# Autodesk Inventor assembly: untitled.brd
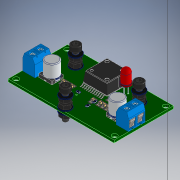
[picture p0: Inventor's stored thumbnail of the model, 180x180]
Saved by Autodesk Inventor 2022 (Build 260153000, 153)
## iProperties
Created: 2022-12-24
Part Number: untitled.brd
Document SubType Name: Assembly
Designer: Ivan Petrov
Author: Ivan Petrov
## Documents named in this file (12)
- C:\Users\Ivan Petrov\Documents\GitHub\OmniBot\design\000.007 - Бортовой источник питания СБ.iam
- C:\Users\Ivan Petrov\Documents\GitHub\OmniBot\design\000.007.001 - Плата печатная.ipt
- C:\Users\Ivan Petrov\Documents\GitHub\OmniBot\design\standart_components\TO-PMOD NDY-11.ipt
- C:\Users\Ivan Petrov\Documents\GitHub\OmniBot\design\standart_components\smd resistors\0R.iam
- C:\Users\Ivan Petrov\Documents\GitHub\OmniBot\design\standart_components\Capacitors smd\Сборка1.iam
- C:\Users\Ivan Petrov\Documents\GitHub\OmniBot\design\standart_components\Capacitors smd\05_NICHICON_8X10_NEWARK_58R3566_ENSAMBLE.ipt
- C:\Users\Ivan Petrov\Documents\GitHub\OmniBot\design\standart_components\LED-Red.ipt
- C:\Users\Ivan Petrov\Documents\GitHub\OmniBot\design\standart_components\Capacitors smd\000.007.002 - Радиатор.ipt
- C:\Users\Ivan Petrov\Documents\GitHub\OmniBot\design\standart_components\Terminal Block 2P.ipt
- C:\Users\Ivan Petrov\Documents\GitHub\OmniBot\design\Content Center Files\ru-RU\DIN 912\DIN 912 - M3 x 0,5 x 16 x 14,75.ipt
- C:\Users\Ivan Petrov\Documents\GitHub\OmniBot\design\Content Center Files\ru-RU\AS 1237 (3.1)\AS 1237 - 3 mm(1)Aluminium-6061.ipt
- C:\Users\Ivan Petrov\Documents\GitHub\OmniBot\design\Content Center Files\ru-RU\AS 1112 (2)\AS 1112 - M3  Тип 5.ipt
## Components (43 placed, 23 different names)
1. untitled.brdКонтур:1 — Совмещение:2, Совмещение:11, Совмещение:20, Совмещение:21, Совмещение:22, Совмещение:23, Совмещение:24, Совмещение:25, Угол:1, Совмещение:26, Угол:2, Вставка:4, Вставка:5, Вставка:6, Вставка:14, Вставка:15, Вставка:16
2. C1_2 [sub-assembly]
3. C2_3 [sub-assembly]
4. C3_4 [sub-assembly]
5. C4_5 [sub-assembly]
6. C5_6 [sub-assembly]
7. C6_7 [sub-assembly]
8. C7_8 [sub-assembly]
9. C8_9 [sub-assembly]
10. R1_24 [sub-assembly]
11. R2_25 [sub-assembly]
12. R3_26 [sub-assembly]
13. R4_27 [sub-assembly]
14. R5_28 [sub-assembly]
15. R6_29 [sub-assembly]
16. TO-PMOD NDY-11:1 — Совмещение:2, Заподлицо:1, Совмещение:27
17. 05_NICHICON_8X10_NEWARK_58R3566_ENSAMBLE:1 — Совмещение:10, Совмещение:11
18. 05_NICHICON_8X10_NEWARK_58R3566_ENSAMBLE:2 — Совмещение:19, Совмещение:20
19. LED-Red:1 — Совмещение:21, Совмещение:22, Заподлицо:1
20. 000.007.002 - Радиатор:1 — Совмещение:27, Вставка:1, Вставка:2, Вставка:3, Вставка:11, Вставка:12, Вставка:13
21. Terminal Block 2P:1 — Совмещение:23, Совмещение:25, Угол:1
22. Terminal Block 2P:2 — Совмещение:24, Совмещение:26, Угол:2
23. DIN 912 - заменено на DIN EN ISO 4762 M3 x 16:1 — Вставка:1
24. DIN 912 - заменено на DIN EN ISO 4762 M3 x 16:2 — Вставка:2
25. DIN 912 - заменено на DIN EN ISO 4762 M3 x 16:3 — Вставка:3
26. AS 1237 (3.1) 3 mm - Алюминий 6061:1 — Вставка:4, Вставка:19
27. AS 1237 (3.1) 3 mm - Алюминий 6061:2 — Вставка:5, Вставка:17
28. AS 1237 (3.1) 3 mm - Алюминий 6061:3 — Вставка:6, Вставка:18
29. AS 1237 (3.1) 3 mm - Алюминий 6061:8 — Вставка:11, Вставка:20
30. AS 1237 (3.1) 3 mm - Алюминий 6061:9 — Вставка:12, Вставка:21
31. AS 1237 (3.1) 3 mm - Алюминий 6061:10 — Вставка:13, Вставка:25
32. AS 1237 (3.1) 3 mm - Алюминий 6061:11 — Вставка:14, Вставка:23
33. AS 1237 (3.1) 3 mm - Алюминий 6061:12 — Вставка:15, Вставка:24
34. AS 1237 (3.1) 3 mm - Алюминий 6061:13 — Вставка:16, Вставка:22
35. AS 1112 (2) - метрическая M3  Тип 5:1 — Вставка:17
36. AS 1112 (2) - метрическая M3  Тип 5:2 — Вставка:18
37. AS 1112 (2) - метрическая M3  Тип 5:3 — Вставка:19
38. AS 1112 (2) - метрическая M3  Тип 5:4 — Вставка:20
39. AS 1112 (2) - метрическая M3  Тип 5:5 — Вставка:21
40. AS 1112 (2) - метрическая M3  Тип 5:6 — Вставка:22
41. AS 1112 (2) - метрическая M3  Тип 5:7 — Вставка:23
42. AS 1112 (2) - метрическая M3  Тип 5:8 — Вставка:24
43. AS 1112 (2) - метрическая M3  Тип 5:9 — Вставка:25
## Relationships (42: Insert 21, Mate 18, Angle 2, Flush 1)
- Совмещение:2 [Mate]: untitled.brdКонтур:1 ↔ TO-PMOD NDY-11:1
- Совмещение:7 [Mate]
- Совмещение:8 [Mate]
- Совмещение:9 [Mate]
- Совмещение:10 [Mate]: 05_NICHICON_8X10_NEWARK_58R3566_ENSAMBLE:1
- Совмещение:11 [Mate]: untitled.brdКонтур:1 ↔ 05_NICHICON_8X10_NEWARK_58R3566_ENSAMBLE:1
- Совмещение:16 [Mate]
- Совмещение:17 [Mate]
- Совмещение:18 [Mate]
- Совмещение:19 [Mate]: 05_NICHICON_8X10_NEWARK_58R3566_ENSAMBLE:2
- Совмещение:20 [Mate]: untitled.brdКонтур:1 ↔ 05_NICHICON_8X10_NEWARK_58R3566_ENSAMBLE:2
- Совмещение:21 [Mate]: untitled.brdКонтур:1 ↔ LED-Red:1
- Совмещение:22 [Mate]: untitled.brdКонтур:1 ↔ LED-Red:1
- Заподлицо:1 [Flush]: TO-PMOD NDY-11:1 ↔ LED-Red:1
- Совмещение:23 [Mate]: untitled.brdКонтур:1 ↔ Terminal Block 2P:1
- Совмещение:24 [Mate]: untitled.brdКонтур:1 ↔ Terminal Block 2P:2
- Совмещение:25 [Mate]: untitled.brdКонтур:1 ↔ Terminal Block 2P:1
- Угол:1 [Angle] (-90 deg): untitled.brdКонтур:1 ↔ Terminal Block 2P:1
- Совмещение:26 [Mate]: untitled.brdКонтур:1 ↔ Terminal Block 2P:2
- Угол:2 [Angle] (0 deg): untitled.brdКонтур:1 ↔ Terminal Block 2P:2
- Совмещение:27 [Mate]: TO-PMOD NDY-11:1 ↔ 000.007.002 - Радиатор:1
- Вставка:1 [Insert]: 000.007.002 - Радиатор:1 ↔ DIN 912 - заменено на DIN EN ISO 4762 M3 x 16:1
- Вставка:2 [Insert]: 000.007.002 - Радиатор:1 ↔ DIN 912 - заменено на DIN EN ISO 4762 M3 x 16:2
- Вставка:3 [Insert]: 000.007.002 - Радиатор:1 ↔ DIN 912 - заменено на DIN EN ISO 4762 M3 x 16:3
- Вставка:4 [Insert]: untitled.brdКонтур:1 ↔ AS 1237 (3.1) 3 mm - Алюминий 6061:1
- Вставка:5 [Insert]: untitled.brdКонтур:1 ↔ AS 1237 (3.1) 3 mm - Алюминий 6061:2
- Вставка:6 [Insert]: untitled.brdКонтур:1 ↔ AS 1237 (3.1) 3 mm - Алюминий 6061:3
- Вставка:11 [Insert]: 000.007.002 - Радиатор:1 ↔ AS 1237 (3.1) 3 mm - Алюминий 6061:8
- Вставка:12 [Insert]: 000.007.002 - Радиатор:1 ↔ AS 1237 (3.1) 3 mm - Алюминий 6061:9
- Вставка:13 [Insert]: 000.007.002 - Радиатор:1 ↔ AS 1237 (3.1) 3 mm - Алюминий 6061:10
- Вставка:14 [Insert]: untitled.brdКонтур:1 ↔ AS 1237 (3.1) 3 mm - Алюминий 6061:11
- Вставка:15 [Insert]: untitled.brdКонтур:1 ↔ AS 1237 (3.1) 3 mm - Алюминий 6061:12
- Вставка:16 [Insert]: untitled.brdКонтур:1 ↔ AS 1237 (3.1) 3 mm - Алюминий 6061:13
- Вставка:17 [Insert]: AS 1237 (3.1) 3 mm - Алюминий 6061:2 ↔ AS 1112 (2) - метрическая M3  Тип 5:1
- Вставка:18 [Insert]: AS 1237 (3.1) 3 mm - Алюминий 6061:3 ↔ AS 1112 (2) - метрическая M3  Тип 5:2
- Вставка:19 [Insert]: AS 1237 (3.1) 3 mm - Алюминий 6061:1 ↔ AS 1112 (2) - метрическая M3  Тип 5:3
- Вставка:20 [Insert]: AS 1237 (3.1) 3 mm - Алюминий 6061:8 ↔ AS 1112 (2) - метрическая M3  Тип 5:4
- Вставка:21 [Insert]: AS 1237 (3.1) 3 mm - Алюминий 6061:9 ↔ AS 1112 (2) - метрическая M3  Тип 5:5
- Вставка:22 [Insert]: AS 1237 (3.1) 3 mm - Алюминий 6061:13 ↔ AS 1112 (2) - метрическая M3  Тип 5:6
- Вставка:23 [Insert]: AS 1237 (3.1) 3 mm - Алюминий 6061:11 ↔ AS 1112 (2) - метрическая M3  Тип 5:7
- Вставка:24 [Insert]: AS 1237 (3.1) 3 mm - Алюминий 6061:12 ↔ AS 1112 (2) - метрическая M3  Тип 5:8
- Вставка:25 [Insert]: AS 1237 (3.1) 3 mm - Алюминий 6061:10 ↔ AS 1112 (2) - метрическая M3  Тип 5:9
